# Autodesk Inventor assembly: mascon-new
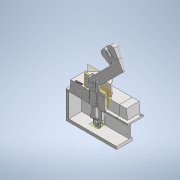
[picture p0: Inventor's stored thumbnail of the model, 180x180]
Saved by Autodesk Inventor 2022 (Build 260153000, 153)
## iProperties
Created: 2021-04-28
Part Number: mascon-new
Document SubType Name: Assembly
Designer: ben
Author: ben
## Documents named in this file (10)
- C:\Users\teh18\OneDrive\BVE Controller\r68-bve-mascon\mascon-new.iam
- C:\Users\teh18\OneDrive\BVE Controller\r68-bve-mascon\handle\handle.iam
- C:\Users\teh18\OneDrive\BVE Controller\r68-bve-mascon\shell\shell.iam
- C:\Users\teh18\OneDrive\BVE Controller\r68-bve-mascon\handle_base_rod.ipt
- C:\Users\teh18\OneDrive\BVE Controller\r68-bve-mascon\handle_holder.ipt
- C:\Users\teh18\OneDrive\BVE Controller\r68-bve-mascon\Reverser.ipt
- C:\Users\teh18\OneDrive\BVE Controller\r68-bve-mascon\handle-base\handle_base.iam
- C:\Users\teh18\OneDrive\BVE Controller\r68-bve-mascon\handle_base2.ipt
- C:\Users\teh18\OneDrive\BVE Controller\r68-bve-mascon\handle-base\PotAttachment.ipt
- C:\Users\teh18\OneDrive\BVE Controller\r68-bve-mascon\handle-base\SpringRod.ipt
## Components (9 placed, 9 different names)
1. shell:1 [sub-assembly] — Flush:4, notch selection
2. handle_base_rod:1 — Flush:11
3. handle_holder:1 — Mate:16
4. Reverser:1 — Flush:4
5. handle:1 [sub-assembly] — Mate:17, Flush:12, Handle Pop
6. handle_base:1 [sub-assembly] — Mate:16, Mate:17, Flush:11, Flush:12, Handle Pop, Mate:25, Mate:26, Mate:27, notch selection
7. handle_base2:1 — Mate:25, Mate:26, Mate:27, Mate:28
8. PotAttachment:1 — Mate:28
9. SpringRod:1
## Relationships (11: Mate 6, Flush 3, RevoluteJoint 2)
- Flush:4: shell:1 ↔ Reverser:1
- Mate:16: handle_holder:1 ↔ handle_base:1
- Mate:17: handle:1 ↔ handle_base:1
- Flush:11: handle_base_rod:1 ↔ handle_base:1
- Flush:12: handle:1 ↔ handle_base:1
- Handle Pop [RevoluteJoint]: handle:1 ↔ handle_base:1
- Mate:25: handle_base:1 ↔ handle_base2:1
- Mate:26: handle_base:1 ↔ handle_base2:1
- Mate:27: handle_base:1 ↔ handle_base2:1
- notch selection [RevoluteJoint]: shell:1 ↔ handle_base:1
- Mate:28: handle_base2:1 ↔ PotAttachment:1
